# Autodesk Inventor assembly: extruder
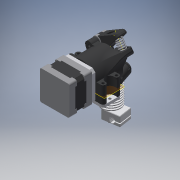
[picture p0: Inventor's stored thumbnail of the model, 180x180]
Saved by Autodesk Inventor 2016 (Build 200138000, 138)
## iProperties
Created: 2016-05-21
Part Number: extruder
Document SubType Name: Assembly
Designer: brent
Author: brent
## Documents named in this file (7)
- C:\Users\brent\OneDrive\personal\printer_cad\extruder\extruder.iam
- C:\Users\brent\OneDrive\personal\printer_cad\extruder\extruder_sketch.ipt
- C:\Users\brent\OneDrive\personal\printer_cad\offtheshelf\gearedstepper.ipt
- C:\Users\brent\OneDrive\personal\printer_cad\offtheshelf\e3dv6.ipt
- C:\Users\brent\OneDrive\personal\printer_cad\offtheshelf\mk8_drivegear.ipt
- C:\Users\brent\OneDrive\personal\printer_cad\offtheshelf\extruder_spring.ipt
- C:\Users\brent\OneDrive\personal\printer_cad\offtheshelf\623bearing.ipt
## Components (8 placed, 6 different names)
1. extruder_sketch:1 — Mate:6, Flush:1, Mate:7, Mate:11, Mate:14, Mate:15, Flush:2, Mate:16, Mate:18, Mate:19, Mate:20, Mate:22, Mate:24, Mate:25, Mate:27, Mate:29, Mate:30, Flush:3
2. gearedstepper:1 — Mate:5, Mate:19, Mate:22, Mate:25, Mate:28
3. e3dv6:1 — Mate:20, Mate:30
4. mk8_drivegear:1 — Mate:5, Mate:6, Mate:28
5. extruder_spring:1 — Flush:1, Mate:7, Mate:15, Flush:2
6. 623bearing:1 — Mate:18, Mate:29
7. 623bearing:2 — Mate:11, Mate:14, Mate:16, Mate:17, Mate:24
8. 623bearing:3 — Mate:17, Mate:27
## Relationships (21: Mate 18, Flush 3)
- Mate:5: gearedstepper:1 ↔ mk8_drivegear:1
- Mate:6 (-3.35 mm): extruder_sketch:1 ↔ mk8_drivegear:1
- Flush:1: extruder_sketch:1 ↔ extruder_spring:1
- Mate:7: extruder_sketch:1 ↔ extruder_spring:1
- Mate:11: extruder_sketch:1 ↔ 623bearing:2
- Mate:14: extruder_sketch:1 ↔ 623bearing:2
- Mate:15: extruder_sketch:1 ↔ extruder_spring:1
- Flush:2: extruder_sketch:1 ↔ extruder_spring:1
- Mate:16: extruder_sketch:1 ↔ 623bearing:2
- Mate:17: 623bearing:2 ↔ 623bearing:3
- Mate:18: extruder_sketch:1 ↔ 623bearing:1
- Mate:19: extruder_sketch:1 ↔ gearedstepper:1
- Mate:20: extruder_sketch:1 ↔ e3dv6:1
- Mate:22: extruder_sketch:1 ↔ gearedstepper:1
- Mate:24: extruder_sketch:1 ↔ 623bearing:2
- Mate:25: extruder_sketch:1 ↔ gearedstepper:1
- Mate:27: extruder_sketch:1 ↔ 623bearing:3
- Mate:28 (1.65 mm): gearedstepper:1 ↔ mk8_drivegear:1
- Mate:29 (0.3 mm): extruder_sketch:1 ↔ 623bearing:1
- Mate:30: extruder_sketch:1 ↔ e3dv6:1
- Flush:3 (10 mm): extruder_sketch:1
